# Autodesk Inventor assembly: endmould_p1
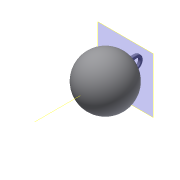
[picture p0: Inventor's stored thumbnail of the model, 180x180]
Saved by Autodesk Inventor 2017 (Build 210142000, 142)
## iProperties
Created: 2018-06-13
Part Number: endmould_p1
Document SubType Name: Assembly
Designer: Nic
Author: Nic
## Documents named in this file (3)
- C:\Users\Nic\Documents\Antenna\endmould_p1.iam
- C:\Users\Nic\Documents\Antenna\end_segment_v2.ipt
- C:\Users\Nic\Documents\Antenna\end_pad.ipt
## Components (2 placed, 2 different names)
1. end_segment_v2:1 — Flush:1, Mate:2
2. end_pad:1 — Flush:1, Mate:1
## Relationships (3: Mate 2, Flush 1)
- Flush:1: end_segment_v2:1 ↔ end_pad:1
- Mate:1: end_pad:1
- Mate:2: end_segment_v2:1
